# Autodesk Inventor assembly: AdditionalLayer
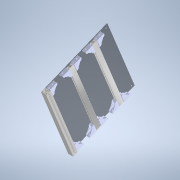
[picture p0: Inventor's stored thumbnail of the model, 180x180]
Saved by Autodesk Inventor 2021.1 (Build 251245010, 245A)
## iProperties
Created: 2020-11-09
Part Number: AdditionalLayer
Document SubType Name: Assembly
Designer: gisen
Author: gisen
## Documents named in this file (5)
- C:\Users\gisen\GitProjects\CAD-Data\CuboidAccessories\SecurityBox\Assemblies\AdditionalLayerAssembly.iam
- C:\Users\gisen\GitProjects\CAD-Data\CuboidAccessories\SecurityBox\Frames\BasicFrameLight290.ipt
- C:\Users\gisen\GitProjects\CAD-Data\GeneralComponentsTemplate\Fittings\BasicFrameBracket.ipt
- C:\Users\gisen\GitProjects\CAD-Data\CuboidAccessories\SecurityBox\Frames\BasicFrameCornerSide290.ipt
- C:\Users\gisen\GitProjects\CAD-Data\CuboidAccessories\SecurityBox\Plates\InsideLayerPlate_290_270.ipt
## Components (14 placed, 4 different names)
1. BasicFrameLight290:1 — メイト:24, フラッシュ:19
2. BasicFrameLight290:2 — フラッシュ:14, フラッシュ:16, フラッシュ:18, メイト:25
3. BasicFrameBracket:1
4. BasicFrameBracket:2 — メイト:19
5. BasicFrameBracket:3
6. BasicFrameBracket:4 — メイト:20
7. BasicFrameBracket:5
8. BasicFrameBracket:6
9. BasicFrameBracket:7
10. BasicFrameBracket:8
11. BasicFrameBracket:9 — フラッシュ:16, メイト:20, メイト:23
12. BasicFrameBracket:10 — フラッシュ:14, メイト:19, メイト:22, フラッシュ:20
13. BasicFrameCornerSide290:1 — フラッシュ:18, メイト:22, メイト:23, フラッシュ:21, メイト:25
14. InsideLayerPlate_290_270:1 — メイト:24, フラッシュ:19, フラッシュ:20, フラッシュ:21
## Relationships (39: Mate 23, Flush 16)
- [Mate] (80 mm): BasicFrameLight290:1 ↔ BasicFrameLight290:2
- [Mate]: BasicFrameLight290:1 ↔ BasicFrameBracket:1
- [Mate]: BasicFrameLight290:1 ↔ BasicFrameBracket:2
- [Mate]: BasicFrameLight290:2 ↔ BasicFrameBracket:5
- [Mate]: BasicFrameLight290:2 ↔ BasicFrameBracket:6
- [Mate]: BasicFrameLight290:1 ↔ BasicFrameBracket:3
- [Mate]: BasicFrameLight290:1 ↔ BasicFrameBracket:4
- [Mate]: BasicFrameLight290:2 ↔ BasicFrameBracket:7
- [Mate]: BasicFrameLight290:2 ↔ BasicFrameBracket:8
- [Flush]: BasicFrameLight290:1 ↔ BasicFrameBracket:1
- [Flush]: BasicFrameLight290:1 ↔ BasicFrameBracket:2
- [Flush]: BasicFrameLight290:1 ↔ BasicFrameBracket:3
- [Flush]: BasicFrameLight290:1 ↔ BasicFrameBracket:4
- [Flush]: BasicFrameLight290:1 ↔ BasicFrameLight290:2
- [Flush]: BasicFrameLight290:2 ↔ BasicFrameBracket:5
- [Flush]: BasicFrameLight290:2 ↔ BasicFrameBracket:6
- [Flush]: BasicFrameLight290:2 ↔ BasicFrameBracket:7
- [Flush]: BasicFrameLight290:2 ↔ BasicFrameBracket:8
- [Mate] (-5 mm): BasicFrameLight290:1 ↔ BasicFrameBracket:4
- [Mate] (-5 mm): BasicFrameLight290:2 ↔ BasicFrameBracket:8
- [Mate] (-5 mm): BasicFrameLight290:2 ↔ BasicFrameBracket:7
- [Mate] (-5 mm): BasicFrameLight290:2 ↔ BasicFrameBracket:5
- [Mate] (-5 mm): BasicFrameLight290:2 ↔ BasicFrameBracket:6
- [Mate] (-5 mm): BasicFrameLight290:1 ↔ BasicFrameBracket:3
- [Mate] (-5 mm): BasicFrameLight290:1 ↔ BasicFrameBracket:1
- [Mate] (-5 mm): BasicFrameLight290:1 ↔ BasicFrameBracket:2
- [Flush]: BasicFrameLight290:1 ↔ BasicFrameLight290:2
- フラッシュ:14 [Flush]: BasicFrameLight290:2 ↔ BasicFrameBracket:10
- フラッシュ:16 [Flush]: BasicFrameLight290:2 ↔ BasicFrameBracket:9
- メイト:19 [Mate]: BasicFrameBracket:2 ↔ BasicFrameBracket:10
- メイト:20 [Mate]: BasicFrameBracket:4 ↔ BasicFrameBracket:9
- フラッシュ:18 [Flush]: BasicFrameLight290:2 ↔ BasicFrameCornerSide290:1
- メイト:22 [Mate]: BasicFrameBracket:10 ↔ BasicFrameCornerSide290:1
- メイト:23 [Mate]: BasicFrameBracket:9 ↔ BasicFrameCornerSide290:1
- メイト:24 [Mate] (2.5 mm): BasicFrameLight290:1 ↔ InsideLayerPlate_290_270:1
- フラッシュ:19 [Flush]: BasicFrameLight290:1 ↔ InsideLayerPlate_290_270:1
- フラッシュ:20 [Flush]: BasicFrameBracket:10 ↔ InsideLayerPlate_290_270:1
- フラッシュ:21 [Flush]: BasicFrameCornerSide290:1 ↔ InsideLayerPlate_290_270:1
- メイト:25 [Mate] (85 mm): BasicFrameLight290:2 ↔ BasicFrameCornerSide290:1
## Named parameters: d338_d324 = 0 mm, d339_d325 = 0 mm, d340_d326 = 0 mm, d341_d327 = 0 mm, d342_d328 = 0 mm, d343_d329 = 0 mm, d344_d330 = 0 mm, d345_d331 = 0 mm, d346_d332 = 0 mm, d347_d224 = 0 mm, d348_d200 = 80 mm, d349_d203 = 0 mm, d350_d205 = 0 mm, d351_d209 = 0 mm, d352_d211 = 0 mm, d353_d214 = 0 mm, d354_d218 = 0 mm, d355_d220 = 0 mm
